# Autodesk Inventor assembly: NC
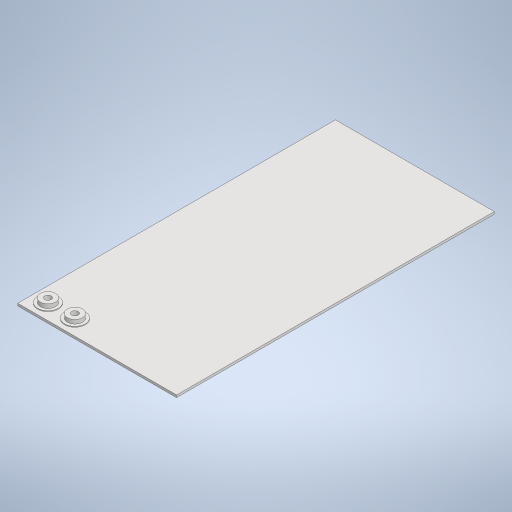
[picture p0: Inventor's stored thumbnail of the model, 512x512]
Saved by Autodesk Inventor 2023 (Build 270158000, 158)
## iProperties
Created: 2022-06-01
Part Number: NC
Document SubType Name: Assembly
Designer: yuta
Author: yuta
## Documents named in this file (3)
- C:\Users\yuta\Documents\NHK\NC\NC.iam
- C:\Users\yuta\Documents\NHK\NC.port.ipt
- C:\Users\yuta\Documents\NHK\新人講習ブッシュベアリング.ipt
## Components (3 placed, 2 different names)
1. NC.port:1 — メイト:2, メイト:3, メイト:4, メイト:5, メイト:6, メイト:7
2. 新人講習ブッシュベアリング:1 — メイト:5, メイト:6, メイト:7
3. 新人講習ブッシュベアリング:2 — メイト:2, メイト:3, メイト:4
## Relationships (6: Mate 6)
- メイト:2 [Mate]: NC.port:1 ↔ 新人講習ブッシュベアリング:2
- メイト:3 [Mate] (-19 mm): NC.port:1 ↔ 新人講習ブッシュベアリング:2
- メイト:4 [Mate] (-19 mm): NC.port:1 ↔ 新人講習ブッシュベアリング:2
- メイト:5 [Mate]: NC.port:1 ↔ 新人講習ブッシュベアリング:1
- メイト:6 [Mate] (-19 mm): NC.port:1 ↔ 新人講習ブッシュベアリング:1
- メイト:7 [Mate] (-53 mm): NC.port:1 ↔ 新人講習ブッシュベアリング:1
